# Autodesk Inventor assembly: 머리 조립품
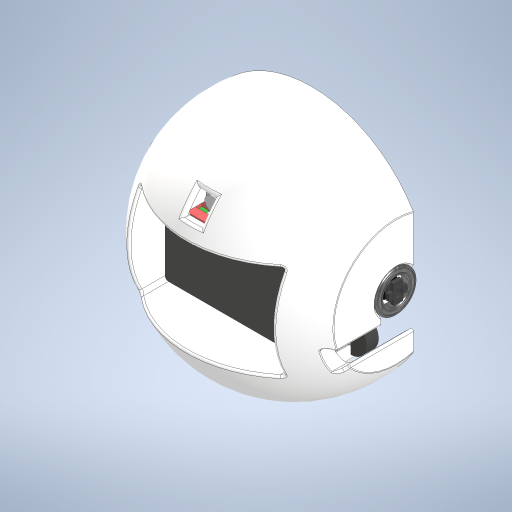
[picture p0: Inventor's stored thumbnail of the model, 512x512]
Saved by Autodesk Inventor 2023 (Build 270158000, 158)
## iProperties
Created: 2022-08-09
Part Number: 머리 조립품
Document SubType Name: Assembly
Designer: fly01
Author: fly01
## Documents named in this file (12)
- C:\Users\user\Desktop\PAI\PAI설계\조림품\머리 조립품.iam
- C:\Users\user\Desktop\PAI\PAI설계\출력품\Head_front.ipt
- C:\Users\user\Desktop\PAI\PAI설계\조림품\라즈베리파이 조립품.iam
- C:\Users\user\Desktop\PAI\PAI설계\출력품\라즈베리파이 고정 커버.ipt
- C:\Users\user\Desktop\PAI\PAI설계\범용 부품\쿨러.ipt
- C:\Users\user\Desktop\PAI\PAI설계\출력품\Head_back.ipt
- C:\Users\user\Desktop\PAI\PAI설계\범용 부품\180도 서보모터.ipt
- C:\Users\user\Desktop\PAI\PAI설계\범용 부품\베어링 6802zz.ipt
- C:\Users\user\Desktop\PAI\PAI설계\범용 부품\베어링 MR84ZZ.ipt
- C:\Users\user\Desktop\PAI\PAI설계\범용 부품\180도 서보모터 십자축 자른 것.ipt
- C:\Users\user\Desktop\PAI\PAI설계\출력품\라즈베리파이 카메라 고정대.ipt
- C:\Users\user\Desktop\PAI\PAI설계\범용 부품\RasCamera.ipt
## Components (11 placed, 11 different names)
1. Head_front:1 — 삽입:8, 삽입:9, 삽입:14, 삽입:15
2. 라즈베리파이 조립품:1 [sub-assembly] — 회전:1
3. 라즈베리파이 고정 커버:1 — 회전:1
4. 쿨러:1
5. Head_back:1
6. 180도 서보모터:1 — 삽입:7, 삽입:8
7. 베어링 6802zz:1 — 삽입:14
8. 베어링 MR84ZZ:1 — 삽입:9
9. 180도 서보모터 십자축 자른 것:1 — 삽입:7
10. 라즈베리파이 카메라 고정대:1 — 삽입:10, 삽입:11, 삽입:15
11. RasCamera:1 — 삽입:10, 삽입:11
## Relationships (8: Insert 7, RevoluteJoint 1)
- 회전:1 [RevoluteJoint]: 라즈베리파이 조립품:1 ↔ 라즈베리파이 고정 커버:1
- 삽입:7 [Insert]: 180도 서보모터:1 ↔ 180도 서보모터 십자축 자른 것:1
- 삽입:8 [Insert]: Head_front:1 ↔ 180도 서보모터:1
- 삽입:9 [Insert]: Head_front:1 ↔ 베어링 MR84ZZ:1
- 삽입:10 [Insert]: 라즈베리파이 카메라 고정대:1 ↔ RasCamera:1
- 삽입:11 [Insert]: 라즈베리파이 카메라 고정대:1 ↔ RasCamera:1
- 삽입:14 [Insert]: Head_front:1 ↔ 베어링 6802zz:1
- 삽입:15 [Insert]: Head_front:1 ↔ 라즈베리파이 카메라 고정대:1
